# Autodesk Inventor assembly: Chasis inferior _1_
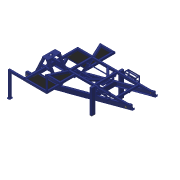
[picture p0: Inventor's stored thumbnail of the model, 180x180]
Saved by Autodesk Inventor 2020 (Build 240168000, 168)
## iProperties
Created: 2020-02-27
Part Number: Chasis inferior _1_
Document SubType Name: Assembly
Designer: Juan Carlos Botero
Author: Juan Carlos Botero
## Documents named in this file (49)
- D:\Drives\OneDrive\Carlos_2\02 TRABAJOS\MULTIPLO\Conveyor\ORIGINAL_RUA\Chasis inferior _1_.iam
- D:\Drives\OneDrive\Carlos_2\02 TRABAJOS\MULTIPLO\Conveyor\ORIGINAL_RUA\Refuerzo diagonal tiro.ipt
- D:\Drives\OneDrive\Carlos_2\02 TRABAJOS\MULTIPLO\Conveyor\ORIGINAL_RUA\Lamina escalon 2.ipt
- D:\Drives\OneDrive\Carlos_2\02 TRABAJOS\MULTIPLO\Conveyor\ORIGINAL_RUA\Lamina sujeción bateria 2.ipt
- D:\Drives\OneDrive\Carlos_2\02 TRABAJOS\MULTIPLO\Conveyor\ORIGINAL_RUA\Refuerzo perfil en C.ipt
- D:\Drives\OneDrive\Carlos_2\02 TRABAJOS\MULTIPLO\Conveyor\ORIGINAL_RUA\Tapa perfil 100x50.ipt
- D:\Drives\OneDrive\Carlos_2\02 TRABAJOS\MULTIPLO\Conveyor\ORIGINAL_RUA\Angulo soporte batería 1.ipt
- D:\Drives\OneDrive\Carlos_2\02 TRABAJOS\MULTIPLO\Conveyor\ORIGINAL_RUA\Perfil 1 en C derecho 2.ipt
- D:\Drives\OneDrive\Carlos_2\02 TRABAJOS\MULTIPLO\Conveyor\ORIGINAL_RUA\Unión vigas chasis.ipt
- D:\Drives\OneDrive\Carlos_2\02 TRABAJOS\MULTIPLO\Conveyor\ORIGINAL_RUA\Caucho tope banda.ipt
- D:\Drives\OneDrive\Carlos_2\02 TRABAJOS\MULTIPLO\Conveyor\ORIGINAL_RUA\Refuerzo diagonal chasis inferior.ipt
- D:\Drives\OneDrive\Carlos_2\02 TRABAJOS\MULTIPLO\Conveyor\ORIGINAL_RUA\Perfil escalón 6.ipt
- D:\Drives\OneDrive\Carlos_2\02 TRABAJOS\MULTIPLO\Conveyor\ORIGINAL_RUA\Perfil escalón 3.ipt
- D:\Drives\OneDrive\Carlos_2\02 TRABAJOS\MULTIPLO\Conveyor\ORIGINAL_RUA\Refuerzo chasis.ipt
- D:\Drives\OneDrive\Carlos_2\02 TRABAJOS\MULTIPLO\Conveyor\ORIGINAL_RUA\Perfil escalón 4.ipt
- D:\Drives\OneDrive\Carlos_2\02 TRABAJOS\MULTIPLO\Conveyor\ORIGINAL_RUA\Tope banda.ipt
- D:\Drives\OneDrive\Carlos_2\02 TRABAJOS\MULTIPLO\Conveyor\ORIGINAL_RUA\Lamina indexacion eje trasero.ipt
- D:\Drives\OneDrive\Carlos_2\02 TRABAJOS\MULTIPLO\Conveyor\ORIGINAL_RUA\Refuerzo horizontal tiro.ipt
- D:\Drives\OneDrive\Carlos_2\02 TRABAJOS\MULTIPLO\Conveyor\ORIGINAL_RUA\Angulo escalón 1.ipt
- D:\Drives\OneDrive\Carlos_2\02 TRABAJOS\MULTIPLO\Conveyor\ORIGINAL_RUA\Base chasis inferior izquierdo.ipt
- D:\Drives\OneDrive\Carlos_2\02 TRABAJOS\MULTIPLO\Conveyor\ORIGINAL_RUA\Refuerzo diagonal estructura tiro.ipt
- D:\Drives\OneDrive\Carlos_2\02 TRABAJOS\MULTIPLO\Conveyor\ORIGINAL_RUA\Perfil 1 en C izquierdo 2.ipt
- D:\Drives\OneDrive\Carlos_2\02 TRABAJOS\MULTIPLO\Conveyor\ORIGINAL_RUA\Lamina escalon 1.ipt
- D:\Drives\OneDrive\Carlos_2\02 TRABAJOS\MULTIPLO\Conveyor\ORIGINAL_RUA\Lamina pivote actuador lineal pequeño.ipt
- D:\Drives\OneDrive\Carlos_2\02 TRABAJOS\MULTIPLO\Conveyor\ORIGINAL_RUA\Perfil 1 en C izquierdo 1.ipt
- D:\Drives\OneDrive\Carlos_2\02 TRABAJOS\MULTIPLO\Conveyor\ORIGINAL_RUA\Perfil 1 en C derecho 1.ipt
- D:\Drives\OneDrive\Carlos_2\02 TRABAJOS\MULTIPLO\Conveyor\ORIGINAL_RUA\Lamina baliza.ipt
- D:\Drives\OneDrive\Carlos_2\02 TRABAJOS\MULTIPLO\Conveyor\ORIGINAL_RUA\Perfil escalón 2.ipt
- D:\Drives\OneDrive\Carlos_2\02 TRABAJOS\MULTIPLO\Conveyor\ORIGINAL_RUA\Perfil escalón 5.ipt
- D:\Drives\OneDrive\Carlos_2\02 TRABAJOS\MULTIPLO\Conveyor\ORIGINAL_RUA\Platina inferior actuador lineal.ipt
- D:\Drives\OneDrive\Carlos_2\02 TRABAJOS\MULTIPLO\Conveyor\ORIGINAL_RUA\Angulo escalón 3.ipt
- D:\Drives\OneDrive\Carlos_2\02 TRABAJOS\MULTIPLO\Conveyor\ORIGINAL_RUA\Perfil escalón 1.ipt
- D:\Drives\OneDrive\Carlos_2\02 TRABAJOS\MULTIPLO\Conveyor\ORIGINAL_RUA\Pie amigo lamina quinta rueda.ipt
- D:\Drives\OneDrive\Carlos_2\02 TRABAJOS\MULTIPLO\Conveyor\ORIGINAL_RUA\Perfil 2 en C derecho.ipt
- D:\Drives\OneDrive\Carlos_2\02 TRABAJOS\MULTIPLO\Conveyor\ORIGINAL_RUA\Perfil 2 en C izquierdo.ipt
- D:\Drives\OneDrive\Carlos_2\02 TRABAJOS\MULTIPLO\Conveyor\ORIGINAL_RUA\Lamina pivote quinta rueda.ipt
- D:\Drives\OneDrive\Carlos_2\02 TRABAJOS\MULTIPLO\Conveyor\ORIGINAL_RUA\Angulo soporte batería 3.ipt
- D:\Drives\OneDrive\Carlos_2\02 TRABAJOS\MULTIPLO\Conveyor\ORIGINAL_RUA\Angulo soporte batería 2.ipt
- D:\Drives\OneDrive\Carlos_2\02 TRABAJOS\MULTIPLO\Conveyor\ORIGINAL_RUA\Unión base chasis inferior.ipt
- D:\Drives\OneDrive\Carlos_2\02 TRABAJOS\MULTIPLO\Conveyor\ORIGINAL_RUA\Soporte baliza.ipt
- D:\Drives\OneDrive\Carlos_2\02 TRABAJOS\MULTIPLO\Conveyor\ORIGINAL_RUA\Base chasis inferior derecho.ipt
- D:\Drives\OneDrive\Carlos_2\02 TRABAJOS\MULTIPLO\Conveyor\ORIGINAL_RUA\Refuerzo intermedio.ipt
- D:\Drives\OneDrive\Carlos_2\02 TRABAJOS\MULTIPLO\Conveyor\ORIGINAL_RUA\Ensamble cuñas y soporte _1_.iam
- D:\Drives\OneDrive\Carlos_2\02 TRABAJOS\MULTIPLO\Conveyor\ORIGINAL_RUA\Espaciador de nylon.ipt
- D:\Drives\OneDrive\Carlos_2\02 TRABAJOS\MULTIPLO\Conveyor\ORIGINAL_RUA\Buje.ipt
- D:\Drives\OneDrive\Carlos_2\02 TRABAJOS\MULTIPLO\Conveyor\ORIGINAL_RUA\Espaciador pivote 1.ipt
- D:\Drives\OneDrive\Carlos_2\02 TRABAJOS\MULTIPLO\Conveyor\ORIGINAL_RUA\Refuerzo diagonal.ipt
- D:\Drives\OneDrive\Carlos_2\02 TRABAJOS\MULTIPLO\Conveyor\ORIGINAL_RUA\Espaciador pivote 2.ipt
- D:\Drives\OneDrive\Carlos_2\02 TRABAJOS\MULTIPLO\Conveyor\ORIGINAL_RUA\Ensamble cuñas y soporte _1__1.iam
## Components (93 placed, 47 different names)
1. Refuerzo diagonal tiro:1
2. Lamina escalon 2:1
3. Lamina sujeción bateria 2:1
4. Refuerzo perfil en C:1
5. Tapa perfil 100x50:1 — Mate:6, Flush:8, Flush:9, Mate:7, Flush:10, Flush:11
6. Angulo soporte batería 1:1
7. Perfil 1 en C derecho 2:1
8. Unión vigas chasis:1
9. Caucho tope banda:1 — Mate:3, Flush:2, Flush:3
10. Refuerzo diagonal chasis inferior:1
11. Perfil escalón 6:1
12. Perfil escalón 3:1
13. Refuerzo chasis:1
14. Perfil escalón 4:1
15. Tope banda:1 — Mate:5, Flush:6, Flush:7, Mate:7, Flush:10, Flush:11, Flush:13, Mate:8, Mate:9
16. Lamina indexacion eje trasero:1
17. Refuerzo horizontal tiro:1
18. Angulo escalón 1:1
19. Base chasis inferior izquierdo:1 — Mate:2, Mate:10
20. Refuerzo diagonal estructura tiro:1
21. Perfil 1 en C izquierdo 2:1
22. Lamina escalon 1:1
23. Lamina pivote actuador lineal pequeño:1
24. Perfil 1 en C izquierdo 1:1
25. Perfil 1 en C derecho 1:1
26. Lamina baliza:1
27. Perfil escalón 2:1
28. Perfil escalón 5:1
29. Platina inferior actuador lineal:1
30. Angulo escalón 3:1
31. Perfil escalón 1:1
32. Pie amigo lamina quinta rueda:1
33. Perfil 2 en C derecho:1
34. Perfil 2 en C izquierdo:1
35. Lamina pivote quinta rueda:1
36. Angulo soporte batería 3:1
37. Angulo soporte batería 2:1
38. Unión base chasis inferior:1
39. Soporte baliza:1
40. Base chasis inferior derecho:1 — Flush:15, Mate:9
41. Refuerzo intermedio:1
42. Ensamble cuñas y soporte <1>:1 [sub-assembly]
43. Lamina escalon 2:2
44. Refuerzo perfil en C:2
45. Espaciador de nylon:1
46. Buje:1
47. Perfil escalón 3:2
48. Buje:2
49. Perfil escalón 3:3
50. Lamina indexacion eje trasero:2
51. Refuerzo horizontal tiro:2
52. Caucho tope banda:2 — Mate:6, Flush:8, Flush:9
53. Refuerzo diagonal tiro:2
54. Tapa perfil 100x50:2 — Mate:3, Flush:2, Flush:3, Mate:4, Flush:4, Flush:5
55. Refuerzo diagonal chasis inferior:2
56. Perfil escalón 5:2
57. Lamina pivote actuador lineal pequeño:2
58. Espaciador pivote 1:1
59. Refuerzo chasis:2
60. Unión vigas chasis:2
61. Perfil escalón 3:4 — Mate:8
62. Espaciador de nylon:2
63. Espaciador pivote 1:2
64. Buje:3
65. Perfil escalón 3:5
66. Refuerzo diagonal:1
67. Espaciador de nylon:3
68. Refuerzo diagonal estructura tiro:2
69. Tapa perfil 100x50:3 — Mate:5, Flush:6, Flush:7, Flush:14, Flush:15
70. Perfil escalón 4:2
71. Espaciador pivote 2:1
72. Refuerzo diagonal:2
73. Angulo escalón 3:2
74. Pie amigo lamina quinta rueda:2
75. Espaciador de nylon:4
76. Platina inferior actuador lineal:2
77. Tope banda:2 — Mate:1, Mate:2, Flush:1, Mate:4, Flush:4, Flush:5, Flush:12, Flush:13, Mate:10
78. Refuerzo chasis:3
79. Tapa perfil 100x50:4 — Mate:1, Flush:1, Flush:12, Flush:14
80. Platina inferior actuador lineal:3
81. Pie amigo lamina quinta rueda:3
82. Espaciador pivote 2:2
83. Perfil escalón 2:2
84. Angulo soporte batería 3:2
85. Buje:4
86. Pie amigo lamina quinta rueda:4
87. Perfil escalón 6:2
88. Lamina escalon 1:2
89. Angulo escalón 1:2
90. Perfil escalón 1:2
91. Refuerzo intermedio:2
92. Platina inferior actuador lineal:4
93. Ensamble cuñas y soporte <1>:2 [sub-assembly]
## Relationships (25: Flush 15, Mate 10)
- Mate:1: Tope banda:2 ↔ Tapa perfil 100x50:4
- Mate:2: Base chasis inferior izquierdo:1 ↔ Tope banda:2
- Flush:1: Tope banda:2 ↔ Tapa perfil 100x50:4
- Mate:3: Caucho tope banda:1 ↔ Tapa perfil 100x50:2
- Flush:2: Caucho tope banda:1 ↔ Tapa perfil 100x50:2
- Flush:3: Caucho tope banda:1 ↔ Tapa perfil 100x50:2
- Mate:4: Tapa perfil 100x50:2 ↔ Tope banda:2
- Flush:4: Tapa perfil 100x50:2 ↔ Tope banda:2
- Flush:5: Tapa perfil 100x50:2 ↔ Tope banda:2
- Mate:5: Tope banda:1 ↔ Tapa perfil 100x50:3
- Flush:6: Tope banda:1 ↔ Tapa perfil 100x50:3
- Flush:7: Tope banda:1 ↔ Tapa perfil 100x50:3
- Mate:6: Tapa perfil 100x50:1 ↔ Caucho tope banda:2
- Flush:8: Tapa perfil 100x50:1 ↔ Caucho tope banda:2
- Flush:9: Tapa perfil 100x50:1 ↔ Caucho tope banda:2
- Mate:7: Tapa perfil 100x50:1 ↔ Tope banda:1
- Flush:10: Tapa perfil 100x50:1 ↔ Tope banda:1
- Flush:11: Tapa perfil 100x50:1 ↔ Tope banda:1
- Flush:12: Tope banda:2 ↔ Tapa perfil 100x50:4
- Flush:13: Tope banda:1 ↔ Tope banda:2
- Mate:8 (482 mm): Tope banda:1 ↔ Perfil escalón 3:4
- Flush:14: Tapa perfil 100x50:3 ↔ Tapa perfil 100x50:4
- Flush:15: Base chasis inferior derecho:1 ↔ Tapa perfil 100x50:3
- Mate:9: Tope banda:1 ↔ Base chasis inferior derecho:1
- Mate:10: Base chasis inferior izquierdo:1 ↔ Tope banda:2
